# Autodesk Inventor assembly: servoHolderConfigAssembly
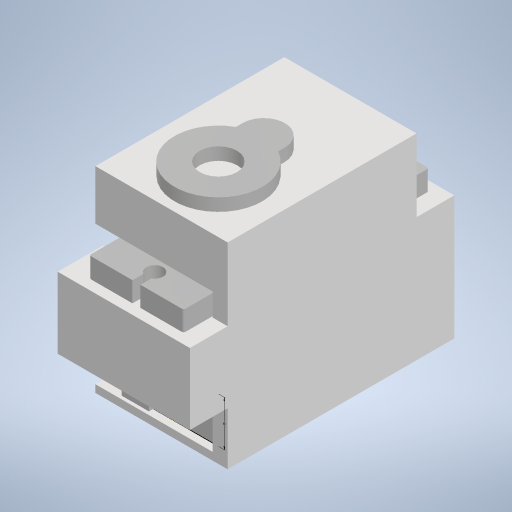
[picture p0: Inventor's stored thumbnail of the model, 512x512]
Saved by Autodesk Inventor 2024 (Build 280153000, 153)
## iProperties
Created: 2024-08-23
Part Number: servoHolderConfigAssembly
Document SubType Name: Assembly
Designer: omiye
Author: omiye
## Documents named in this file (3)
- C:\Projects\Arduino\hexapod\legModels\servoHolderConfigAssembly.iam
- C:\Projects\Arduino\hexapod\legModels\servoHolderBase.ipt
- C:\Users\omiye\Downloads\download\servo v1\servo.ipt
## Components (2 placed, 2 different names)
1. servoHolderBase:1 — Mate:1, Mate:2
2. servo:1 — Mate:1, Mate:2
## Relationships (2: Mate 2)
- Mate:1: servoHolderBase:1 ↔ servo:1
- Mate:2: servoHolderBase:1 ↔ servo:1
